# Autodesk Inventor assembly: pulley asse
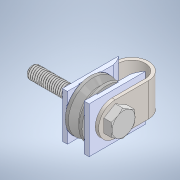
[picture p0: Inventor's stored thumbnail of the model, 180x180]
Saved by Autodesk Inventor 2020.1 (Build 241239000, 239)
## iProperties
Created: 2020-03-07
Part Number: pulley asse
Document SubType Name: Assembly
Designer: Vedant Thorat
Author: Vedant Thorat
## Documents named in this file (5)
- C:\Users\Vedant Thorat\Desktop\pulley\pulley asse.iam
- C:\Users\Vedant Thorat\Desktop\pulley\cover.ipt
- C:\Users\Vedant Thorat\Desktop\pulley\REV-41-1124.ipt
- C:\Users\Vedant Thorat\Desktop\pulley\REV-41-1368.ipt
- C:\Users\Vedant Thorat\Desktop\pulley\buffer.ipt
## Components (5 placed, 4 different names)
1. cover:1 — Insert:1, Insert:2, Insert:3
2. REV-41-1124:1 — Insert:1
3. REV-41-1368:1 — Insert:4
4. buffer:1 — Insert:2, Flush:1, Insert:4
5. buffer:2 — Insert:3, Flush:1
## Relationships (5: Insert 4, Flush 1)
- Insert:1: cover:1 ↔ REV-41-1124:1
- Insert:2: cover:1 ↔ buffer:1
- Insert:3: cover:1 ↔ buffer:2
- Flush:1: buffer:1 ↔ buffer:2
- Insert:4: REV-41-1368:1 ↔ buffer:1
